# Autodesk Inventor assembly: Assembly
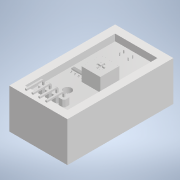
[picture p0: Inventor's stored thumbnail of the model, 180x180]
Saved by Autodesk Inventor 2020 (Build 240168000, 168)
## iProperties
Created: 2019-07-08
Part Number: Assembly
Document SubType Name: Assembly
Designer: simon
Author: simon
## Documents named in this file (3)
- Z:\Dropbox\Coding\3dprint\projects\TCRT5000_Ferraris\Assembly.iam
- Z:\Dropbox\Coding\3dprint\projects\TCRT5000_Ferraris\Holder.ipt
- Z:\Dropbox\Coding\3dprint\projects\TCRT5000_Ferraris\Imported Components\TCRT5000\TCRT5000.ipt
## Components (2 placed, 2 different names)
1. Holder:1 — Mate:1, Mate:2, Mate:3
2. TCRT5000:1 — Mate:1, Mate:2, Mate:3
## Relationships (3: Mate 3)
- Mate:1: Holder:1 ↔ TCRT5000:1
- Mate:2 (1 mm): Holder:1 ↔ TCRT5000:1
- Mate:3 (1 mm): Holder:1 ↔ TCRT5000:1
